# Autodesk Inventor assembly: RT_MAIN_A_001_V0
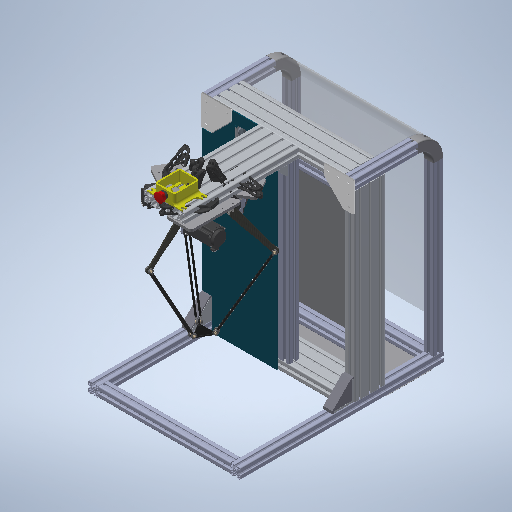
[picture p0: Inventor's stored thumbnail of the model, 512x512]
Saved by Autodesk Inventor 2025.3 (Build 293356000, 356)
## iProperties
Created: 2026-05-15
Part Number: RT_MAIN_A_001_V0
Document SubType Name: Assembly
Designer: louis
Mass: 34530.7 g
Surface Area: 112620 cm^2
Volume: 12343.4 cm^3
Density: 2.7975 g/cm^3
Author: louis
## Documents named in this file (8)
- C:\Users\louis\OneDrive\Desktop\R_Trident\02_CAD\05_Top_Assembly\RT_MAIN_A_001_V0.iam
- C:\Users\louis\OneDrive\Desktop\R_Trident\02_CAD\04_Subassemblies\RT_FRM_A_002_Dynamics.iam
- C:\Users\louis\OneDrive\Desktop\R_Trident\02_CAD\04_Subassemblies\RT_FRM_A_003_FrameV3.iam
- C:\Users\louis\OneDrive\Desktop\R_Trident\02_CAD\04_Subassemblies\RT_ELE_001_ElectricalMainPlate.iam
- C:\Users\louis\OneDrive\Desktop\R_Trident\02_CAD\04_Subassemblies\RT_FRM_A_Left_Front_Cover.iam
- C:\Users\louis\OneDrive\Desktop\R_Trident\02_CAD\03_Parts_Custom\RT_FRM_MC_015_BottomCover.ipt
- C:\Users\louis\OneDrive\Desktop\R_Trident\02_CAD\03_Parts_Custom\RT_FRM_MC_012_Electrical_housing_door.ipt
- C:\Users\louis\OneDrive\Desktop\R_Trident\02_CAD\04_Subassemblies\RT_ELE_A_006_ESTOP.iam
## Components (7 placed, 7 different names)
1. RT_FRM_A_002_Dynamics:1 [sub-assembly] — Mate:20, Mate:21, Mate:22, Flush:6
2. RT_FRM_A_003_FrameV3:1 [sub-assembly] — Flush:5, Mate:22, Flush:6, Mate:23, Flush:7, Mate:25, Flush:8, Flush:9, Flush:10, Flush:11, Flush:12, Mate:26, Flush:13, Mate:27, Flush:14, Flush:15, Flush:16
3. RT_ELE_001_ElectricalMainPlate:1 [sub-assembly] — Mate:23, Mate:24, Flush:7
4. RT_FRM_A_Left_Front_Cover:1 [sub-assembly] — Mate:25, Flush:8, Flush:9
5. RT_FRM_MC_015_BottomCover:1 — Flush:11, Flush:12, Mate:26
6. RT_FRM_MC_012_Electrical_housing_door:1 — Flush:13, Mate:27, Flush:14
7. RT_ELE_A_006_ESTOP:1 [sub-assembly] — Flush:15, Mate:28, Flush:16
## Relationships (23: Flush 12, Mate 11)
- Mate:20: RT_FRM_A_002_Dynamics:1
- Mate:21: RT_FRM_A_002_Dynamics:1
- Mate:16
- Mate:17
- Flush:5: RT_FRM_A_003_FrameV3:1
- Mate:22: RT_FRM_A_002_Dynamics:1 ↔ RT_FRM_A_003_FrameV3:1
- Flush:6 (-300 mm): RT_FRM_A_002_Dynamics:1 ↔ RT_FRM_A_003_FrameV3:1
- Mate:23: RT_FRM_A_003_FrameV3:1 ↔ RT_ELE_001_ElectricalMainPlate:1
- Mate:24: RT_ELE_001_ElectricalMainPlate:1
- Flush:7: RT_FRM_A_003_FrameV3:1 ↔ RT_ELE_001_ElectricalMainPlate:1
- Mate:25: RT_FRM_A_003_FrameV3:1 ↔ RT_FRM_A_Left_Front_Cover:1
- Flush:8 (-1 mm): RT_FRM_A_003_FrameV3:1 ↔ RT_FRM_A_Left_Front_Cover:1
- Flush:9 (-1 mm): RT_FRM_A_003_FrameV3:1 ↔ RT_FRM_A_Left_Front_Cover:1
- Flush:10: RT_FRM_A_003_FrameV3:1
- Flush:11: RT_FRM_A_003_FrameV3:1 ↔ RT_FRM_MC_015_BottomCover:1
- Flush:12: RT_FRM_A_003_FrameV3:1 ↔ RT_FRM_MC_015_BottomCover:1
- Mate:26: RT_FRM_A_003_FrameV3:1 ↔ RT_FRM_MC_015_BottomCover:1
- Flush:13: RT_FRM_A_003_FrameV3:1 ↔ RT_FRM_MC_012_Electrical_housing_door:1
- Mate:27: RT_FRM_A_003_FrameV3:1 ↔ RT_FRM_MC_012_Electrical_housing_door:1
- Flush:14: RT_FRM_A_003_FrameV3:1 ↔ RT_FRM_MC_012_Electrical_housing_door:1
- Flush:15: RT_FRM_A_003_FrameV3:1 ↔ RT_ELE_A_006_ESTOP:1
- Mate:28: RT_ELE_A_006_ESTOP:1
- Flush:16: RT_FRM_A_003_FrameV3:1 ↔ RT_ELE_A_006_ESTOP:1
